# Autodesk Inventor assembly: ASY PRS 9690 Filter legs D1200 940
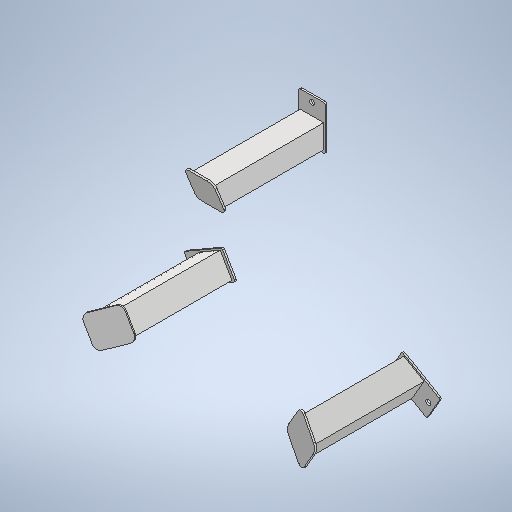
[picture p0: Inventor's stored thumbnail of the model, 512x512]
Saved by Autodesk Inventor 2026.2 (Build 302298000, 298)
## iProperties
Created: 2025-02-20
Part Number: ASY PRS 9690 Filter legs D1200 940
Document SubType Name: Assembly
Designer: admin
Mass: 20950.1 g
Surface Area: 14148.6 cm^2
Volume: 2651.55 cm^3
Density: 7.9011 g/cm^3
Author: user
## Documents named in this file (9)
- C:\Users\admin\Documents\Inventor\PRS-Purovsk\ASY PRS 9690 Filter legs D1200 940.iam
- C:\Users\admin\Documents\Inventor\PRS-Purovsk\PRS 9693 leg sketch_D1200 940.ipt
- C:\Users\admin\Documents\Inventor\PRS-Purovsk\PRS 9681 leg tube_D1200 940.ipt
- C:\Users\admin\Documents\Inventor\PRS-Purovsk\PRS 9785 leg floor channel_D1200 940.ipt
- C:\Users\admin\Documents\Inventor\PRS-Purovsk\PRS 9695 leg floor plate_D1200 940.ipt
- C:\Users\admin\Documents\Inventor\PRS-Purovsk\PRS 9694 leg plate for filter_D1200 940.ipt
- C:\Users\admin\Documents\Inventor\PRS-Purovsk\cc\en-US\ISO 4018\ISO 4018 - M16 x 40.ipt
- C:\Users\admin\Documents\Inventor\PRS-Purovsk\cc\en-US\ISO 7089\ISO 7089 - 16 - 140 HV(1).ipt
- C:\Users\admin\Documents\Inventor\PRS-Purovsk\cc\en-US\ISO 4032(2)\ISO 4032 - M16 - ISO.ipt
## Components (22 placed, 8 different names)
1. PRS 9693 leg sketch_D1200 940:1 — Mate:12
2. ISO 4018 M16 x 40:1 — Mate:15, Mate:14
3. ISO 7089 16:1 — Insert:1, Mate:21, Mate:20
4. ISO 4032 M16:1 — Insert:1
5. ISO 4018 M16 x 40:2 — Mate:17, Mate:16
6. ISO 4018 M16 x 40:3 — Mate:18, Mate:19
7. ISO 7089 16:2 — Insert:2, Mate:23, Mate:22
8. ISO 7089 16:3 — Mate:24, Insert:3, Mate:25
9. ISO 4032 M16:2 — Insert:2
10. ISO 4032 M16:3 — Insert:3
11. PRS 9681 leg tube_D1200 940:1 — Mate:13, Mate:12, Mate:10, Mate:9, Mate:8, Flush:1, Mate:7
12. PRS 9785 leg floor channel_D1200 940:1 — Mate:1, Mate:2, Rigid:10
13. PRS 9695 leg floor plate_D1200 940:1 — Mate:8, Flush:1, Mate:7, Mate:18, Mate:24, Rigid:10
14. PRS 9694 leg plate for filter_D1200 940:1 — Mate:13, Mate:10, Mate:9
15. PRS 9681 leg tube_D1200 940:2
16. PRS 9785 leg floor channel_D1200 940:2 — Mate:21, Mate:23, Mate:25
17. PRS 9695 leg floor plate_D1200 940:2 — Mate:15, Mate:14, Mate:20, Mate:17, Mate:19
18. PRS 9694 leg plate for filter_D1200 940:2
19. PRS 9681 leg tube_D1200 940:3
20. PRS 9785 leg floor channel_D1200 940:3
21. PRS 9695 leg floor plate_D1200 940:3 — Mate:16, Mate:22
22. PRS 9694 leg plate for filter_D1200 940:3
## Component patterns: (3 elements, first: PRS 9681 leg tube_D1200 940:1 + PRS 9785 leg floor channel_D1200 940:1 + PRS 9695 leg floor plate_D1200 940:1 + PRS 9694 leg plate for filter_D1200 940:1)
## Relationships (25: Mate 20, Insert 3, Flush 1, WeldJoint 1)
- Mate:1: PRS 9785 leg floor channel_D1200 940:1
- Mate:2: PRS 9785 leg floor channel_D1200 940:1
- Mate:13: PRS 9681 leg tube_D1200 940:1 ↔ PRS 9694 leg plate for filter_D1200 940:1
- Mate:12: PRS 9693 leg sketch_D1200 940:1 ↔ PRS 9681 leg tube_D1200 940:1
- Mate:10: PRS 9681 leg tube_D1200 940:1 ↔ PRS 9694 leg plate for filter_D1200 940:1
- Mate:9: PRS 9681 leg tube_D1200 940:1 ↔ PRS 9694 leg plate for filter_D1200 940:1
- Mate:8: PRS 9681 leg tube_D1200 940:1 ↔ PRS 9695 leg floor plate_D1200 940:1
- Flush:1 (-10 mm): PRS 9681 leg tube_D1200 940:1 ↔ PRS 9695 leg floor plate_D1200 940:1
- Mate:7: PRS 9681 leg tube_D1200 940:1 ↔ PRS 9695 leg floor plate_D1200 940:1
- Insert:1: ISO 7089 16:1 ↔ ISO 4032 M16:1
- Mate:18: ISO 4018 M16 x 40:3 ↔ PRS 9695 leg floor plate_D1200 940:1
- Mate:24: ISO 7089 16:3 ↔ PRS 9695 leg floor plate_D1200 940:1
- Insert:2: ISO 7089 16:2 ↔ ISO 4032 M16:2
- Insert:3: ISO 7089 16:3 ↔ ISO 4032 M16:3
- Rigid:10 [WeldJoint]: PRS 9785 leg floor channel_D1200 940:1 ↔ PRS 9695 leg floor plate_D1200 940:1
- Mate:15: ISO 4018 M16 x 40:1 ↔ PRS 9695 leg floor plate_D1200 940:2
- Mate:14: ISO 4018 M16 x 40:1 ↔ PRS 9695 leg floor plate_D1200 940:2
- Mate:21: ISO 7089 16:1 ↔ PRS 9785 leg floor channel_D1200 940:2
- Mate:20: ISO 7089 16:1 ↔ PRS 9695 leg floor plate_D1200 940:2
- Mate:17: ISO 4018 M16 x 40:2 ↔ PRS 9695 leg floor plate_D1200 940:2
- Mate:16: ISO 4018 M16 x 40:2 ↔ PRS 9695 leg floor plate_D1200 940:3
- Mate:19: ISO 4018 M16 x 40:3 ↔ PRS 9695 leg floor plate_D1200 940:2
- Mate:23: ISO 7089 16:2 ↔ PRS 9785 leg floor channel_D1200 940:2
- Mate:22: ISO 7089 16:2 ↔ PRS 9695 leg floor plate_D1200 940:3
- Mate:25: ISO 7089 16:3 ↔ PRS 9785 leg floor channel_D1200 940:2
## Named parameters: Out_diam = 963 mm
